# Autodesk Inventor assembly: Main
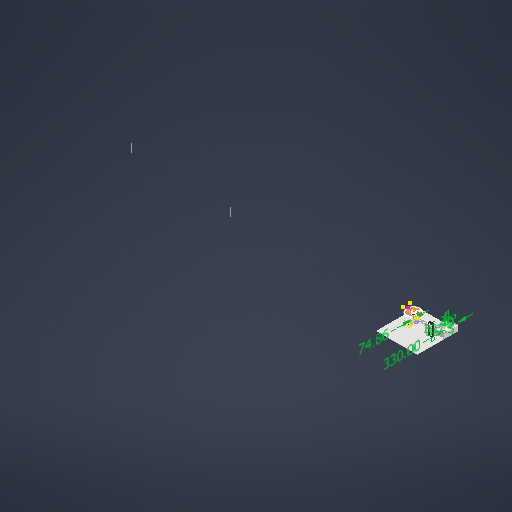
[picture p0: Inventor's stored thumbnail of the model, 512x512]
Saved by Autodesk Inventor 2026.2 (Build 302298000, 298)
## iProperties
Created: 2026-03-06
Part Number: Main
Document SubType Name: Assembly
Designer: danda
Author: danda
## Documents named in this file (13)
- C:\Users\danda\BOM-project\Project\CAD\Main.iam
- C:\Users\danda\BOM-project\Project\CAD\baseb.ipt
- C:\Users\danda\BOM-project\Project\CAD\sorting\Assembly2.iam
- C:\Users\danda\BOM-project\Project\CAD\5mmhieght.ipt
- C:\Users\danda\BOM-project\Project\CAD\collectingslide.ipt
- C:\Users\danda\BOM-project\Project\CAD\newcollection.ipt
- C:\Users\danda\BOM-project\Project\CAD\Lifting\Lifting Mechanism\Assembly2.iam
- C:\Users\danda\BOM-project\Project\CAD\collectionslideintoscrew.ipt
- C:\Users\danda\BOM-project\Project\CAD\outlifting.ipt
- C:\Users\danda\Downloads\ir-sensor-7.snapshot.2\IRsensorhub.ipt
- C:\Users\danda\Downloads\ir-sensor-7.snapshot.2\IRsensors\IRsensors\IRsensors.iam
- C:\Users\danda\BOM-project\Project\CAD\Shooting\Shooting Mechanism Assembly FINAL 2.iam
- C:\Users\danda\BOM-project\Project\CAD\storrageout.ipt
## Components (12 placed, 11 different names)
1. baseb:1 — Mate:1, Mate:2, Mate:3, Mate:9, Flush:3, Flush:4, Mate:21, Mate:22, Mate:24, Mate:41, Mate:44, Mate:45, Flush:11
2. Assembly2:3 [sub-assembly] — Mate:24, Flush:12, Mate:46, Flush:13, Flush:14, Mate:47, Mate:48
3. 5mmhieght:1 — Mate:9, Flush:1, Mate:18, Flush:2
4. collectingslide:1 — Flush:5, Mate:19, Mate:20, Flush:6, Mate:41
5. newcollection:1 — Flush:1, Mate:18, Flush:2, Flush:3, Flush:4, Flush:5, Mate:19
6. Assembly2:4 [sub-assembly] — Mate:22, Flush:7, Mate:23, Flush:10, Mate:42
7. collectionslideintoscrew:1 — Mate:20, Flush:6, Mate:21, Flush:7, Mate:23
8. outlifting:1 — Flush:10, Mate:27, Mate:28, Mate:29, Mate:42, Mate:46, Flush:13, Flush:14
9. IRsensorhub:1 — Mate:27, Mate:28, Mate:29, Mate:30, Mate:31, Mate:32
10. IRsensors:1 [sub-assembly] — Mate:30, Mate:31, Mate:32
11. Shooting Mechanism Assembly FINAL 2:1 [sub-assembly] — Mate:44, Mate:45, Flush:11
12. storrageout:1 — Flush:12, Mate:47, Mate:48
## Relationships (36: Mate 24, Flush 12)
- Mate:1: baseb:1
- Mate:2: baseb:1
- Mate:3: baseb:1
- Mate:9: baseb:1 ↔ 5mmhieght:1
- Flush:1: 5mmhieght:1 ↔ newcollection:1
- Mate:18: 5mmhieght:1 ↔ newcollection:1
- Flush:2: 5mmhieght:1 ↔ newcollection:1
- Flush:3: baseb:1 ↔ newcollection:1
- Flush:4: baseb:1 ↔ newcollection:1
- Flush:5: collectingslide:1 ↔ newcollection:1
- Mate:19: collectingslide:1 ↔ newcollection:1
- Mate:20: collectingslide:1 ↔ collectionslideintoscrew:1
- Flush:6: collectingslide:1 ↔ collectionslideintoscrew:1
- Mate:21: baseb:1 ↔ collectionslideintoscrew:1
- Mate:22: baseb:1 ↔ Assembly2:4
- Flush:7: Assembly2:4 ↔ collectionslideintoscrew:1
- Mate:23: Assembly2:4 ↔ collectionslideintoscrew:1
- Mate:24: baseb:1 ↔ Assembly2:3
- Flush:10: Assembly2:4 ↔ outlifting:1
- Mate:27: outlifting:1 ↔ IRsensorhub:1
- Mate:28: outlifting:1 ↔ IRsensorhub:1
- Mate:29: outlifting:1 ↔ IRsensorhub:1
- Mate:30: IRsensorhub:1 ↔ IRsensors:1
- Mate:31: IRsensorhub:1 ↔ IRsensors:1
- Mate:32: IRsensorhub:1 ↔ IRsensors:1
- Mate:41: baseb:1 ↔ collectingslide:1
- Mate:42: Assembly2:4 ↔ outlifting:1
- Mate:44: baseb:1 ↔ Shooting Mechanism Assembly FINAL 2:1
- Mate:45: baseb:1 ↔ Shooting Mechanism Assembly FINAL 2:1
- Flush:11 (-50 mm): baseb:1 ↔ Shooting Mechanism Assembly FINAL 2:1
- Flush:12: Assembly2:3 ↔ storrageout:1
- Mate:46: Assembly2:3 ↔ outlifting:1
- Flush:13: Assembly2:3 ↔ outlifting:1
- Flush:14: Assembly2:3 ↔ outlifting:1
- Mate:47: Assembly2:3 ↔ storrageout:1
- Mate:48: Assembly2:3 ↔ storrageout:1
